# Autodesk Inventor assembly: Shaft adapter 2
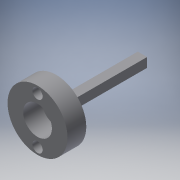
[picture p0: Inventor's stored thumbnail of the model, 180x180]
Saved by Autodesk Inventor 2019 (Build 230136000, 136)
## iProperties
Created: 2019-10-15
Part Number: Shaft adapter 2
Document SubType Name: Assembly
Designer: User
Author: User
## Documents named in this file (3)
- C:\Robotics\CAD\2019-20_CAD\Collection\Shaft adapter 2.iam
- C:\Robotics\CAD\2019-20_CAD\Collection\shaft adapter.ipt
- C:\Robotics\CAD\2019-20_CAD\Collection\Axle part for intake.ipt
## Components (2 placed, 2 different names)
1. shaft adapter:1 — Flush:1, Mate:1, Mate:2
2. Axle part for intake:1 — Flush:1, Mate:1, Mate:2
## Relationships (3: Mate 2, Flush 1)
- Flush:1: shaft adapter:1 ↔ Axle part for intake:1
- Mate:1: shaft adapter:1 ↔ Axle part for intake:1
- Mate:2: shaft adapter:1 ↔ Axle part for intake:1
